# Autodesk Inventor assembly: Workshop_Robot
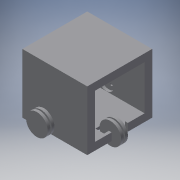
[picture p0: Inventor's stored thumbnail of the model, 180x180]
Saved by Autodesk Inventor 2016 (Build 200138000, 138)
## iProperties
Created: 2016-02-28
Part Number: Workshop_Robot
Document SubType Name: Assembly
Designer: torti_000
Author: torti_000
## Documents named in this file (8)
- C:\Users\torti_000\Documents\Inventor Documents\Workshop_Robot.iam
- C:\Users\torti_000\Documents\Inventor Documents\Bottom_chasis.ipt
- C:\Users\torti_000\Documents\Inventor Documents\Front_chasis.ipt
- C:\Users\torti_000\Documents\Inventor Documents\Side_chasis.ipt
- C:\Users\torti_000\Documents\Inventor Documents\BAck_chasis.ipt
- C:\Users\torti_000\Documents\Inventor Documents\Top_chasis.ipt
- C:\Users\torti_000\Documents\Inventor Documents\Drive_Wheel.ipt
- C:\Users\torti_000\Documents\Inventor Documents\Wheel_design.ipt
## Components (9 placed, 7 different names)
1. Bottom_chasis:1 — Mate:1, Mate:2, Mate:3, Mate:4, Mate:7, Mate:8
2. Front_chasis:1 — Mate:1, Mate:2, Mate:3, Mate:5, Mate:6
3. Side_chasis:1 — Mate:4, Mate:5, Mate:9, Mate:10
4. Side_chasis:2 — Mate:6, Mate:7
5. BAck_chasis:1 — Mate:8, Mate:9, Mate:11
6. Top_chasis:1 — Mate:10, Mate:11
7. Drive_Wheel:1
8. Drive_Wheel:2
9. Wheel_design:1
## Relationships (11: Mate 11)
- Mate:1: Bottom_chasis:1 ↔ Front_chasis:1
- Mate:2: Bottom_chasis:1 ↔ Front_chasis:1
- Mate:3: Bottom_chasis:1 ↔ Front_chasis:1
- Mate:4: Bottom_chasis:1 ↔ Side_chasis:1
- Mate:5: Front_chasis:1 ↔ Side_chasis:1
- Mate:6: Front_chasis:1 ↔ Side_chasis:2
- Mate:7: Bottom_chasis:1 ↔ Side_chasis:2
- Mate:8: Bottom_chasis:1 ↔ BAck_chasis:1
- Mate:9: Side_chasis:1 ↔ BAck_chasis:1
- Mate:10: Side_chasis:1 ↔ Top_chasis:1
- Mate:11: BAck_chasis:1 ↔ Top_chasis:1
